# Autodesk Inventor assembly: frame TOPLEVEL
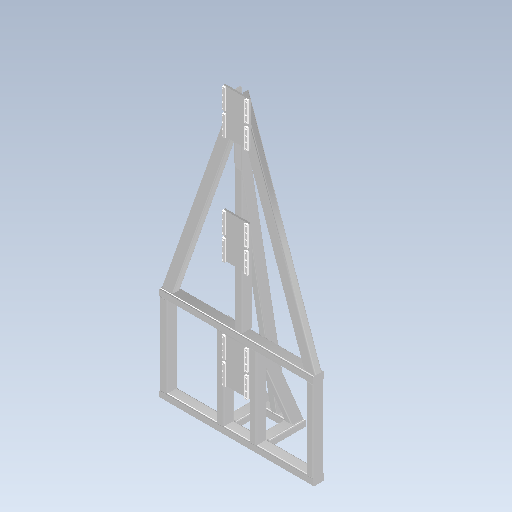
[picture p0: Inventor's stored thumbnail of the model, 512x512]
Saved by Autodesk Inventor 2021 (Build 250183000, 183)
## iProperties
Created: 2021-03-29
Part Number: frame TOPLEVEL
Document SubType Name: Assembly
Designer: Work
Author: Work
## Documents named in this file (12)
- C:\Users\Work\OneDrive - Brookhaven National Laboratory\Daniels, William intern HPR station\Frame\frame TOPLEVEL.iam
- C:\Users\Work\OneDrive - Brookhaven National Laboratory\Daniels, William intern HPR station\Frame\base bar.ipt
- C:\Users\Work\OneDrive - Brookhaven National Laboratory\Daniels, William intern HPR station\Frame\end cap.ipt
- C:\Users\Work\OneDrive - Brookhaven National Laboratory\Daniels, William intern HPR station\Frame\actuMount.iam
- C:\Users\Work\OneDrive - Brookhaven National Laboratory\Daniels, William intern HPR station\Frame\vertical bar.ipt
- C:\Users\Work\OneDrive - Brookhaven National Laboratory\Daniels, William intern HPR station\Frame\depth bar.ipt
- C:\Users\Work\OneDrive - Brookhaven National Laboratory\Daniels, William intern HPR station\Frame\back bar.ipt
- C:\Users\Work\OneDrive - Brookhaven National Laboratory\Daniels, William intern HPR station\Frame\support 1.ipt
- C:\Users\Work\OneDrive - Brookhaven National Laboratory\Daniels, William intern HPR station\Frame\support 2.ipt
- C:\Users\Work\OneDrive - Brookhaven National Laboratory\Daniels, William intern HPR station\Frame\vert support.ipt
- C:\Users\Work\OneDrive - Brookhaven National Laboratory\Daniels, William intern HPR station\Frame\side support.ipt
- C:\Users\Work\OneDrive - Brookhaven National Laboratory\Daniels, William intern HPR station\dimensions.xlsx
## Components (22 placed, 10 different names)
1. base bar:1 — Rigid:1, Rigid:2, Slider:1, Slider:2
2. end cap:1 — Rigid:1, Rigid:3
3. end cap:2 — Rigid:2, Rigid:4
4. actuMount:1 [sub-assembly] — Mate:1, Mate:2, Flush:1, Rigid:11, Rigid:13
5. vertical bar:1 — Rigid:3, Rigid:5
6. vertical bar:2 — Slider:1, Rigid:8, Mate:4, Flush:2
7. vertical bar:3 — Slider:2, Mate:2, Rigid:9, Mate:6, Flush:3
8. vertical bar:4 — Rigid:4, Rigid:6
9. end cap:3 — Rigid:5
10. end cap:4 — Rigid:6, Rigid:7, Mate:12
11. base bar:2 — Rigid:7, Mate:1, Flush:1, Mate:9
12. depth bar:1 — Rigid:8, Rigid:10, Mate:3
13. depth bar:2 — Rigid:9, Mate:5
14. back bar:1 — Rigid:10
15. support 1:1 — Mate:3, Mate:4, Flush:2
16. support 1:2 — Mate:5, Mate:6, Flush:3
17. support 2:1 — Rigid:12, Mate:8, Flush:4, Mate:10, Mate:13
18. actuMount:2 [sub-assembly] — Rigid:11, Rigid:12, Mate:11, Mate:14
19. actuMount:3 [sub-assembly] — Rigid:13, Mate:7
20. vert support:1 — Mate:7, Mate:8, Flush:4
21. side support:1 — Mate:12, Mate:13, Mate:14
22. side support:2 — Mate:9, Mate:10, Mate:11
## Relationships (33: Mate 14, WeldJoint 13, Flush 4, TranslationJoint 2)
- Rigid:1 [WeldJoint]: base bar:1 ↔ end cap:1
- Rigid:2 [WeldJoint]: base bar:1 ↔ end cap:2
- Rigid:3 [WeldJoint]: end cap:1 ↔ vertical bar:1
- Rigid:4 [WeldJoint]: end cap:2 ↔ vertical bar:4
- Slider:1 [TranslationJoint]: base bar:1 ↔ vertical bar:2
- Slider:2 [TranslationJoint]: base bar:1 ↔ vertical bar:3
- Rigid:5 [WeldJoint]: vertical bar:1 ↔ end cap:3
- Rigid:6 [WeldJoint]: vertical bar:4 ↔ end cap:4
- Rigid:7 [WeldJoint]: end cap:4 ↔ base bar:2
- Mate:1: actuMount:1 ↔ base bar:2
- Mate:2: actuMount:1 ↔ vertical bar:3
- Flush:1: actuMount:1 ↔ base bar:2
- Rigid:8 [WeldJoint]: vertical bar:2 ↔ depth bar:1
- Rigid:9 [WeldJoint]: vertical bar:3 ↔ depth bar:2
- Rigid:10 [WeldJoint]: depth bar:1 ↔ back bar:1
- Mate:3: depth bar:1 ↔ support 1:1
- Mate:4: vertical bar:2 ↔ support 1:1
- Flush:2: vertical bar:2 ↔ support 1:1
- Mate:5: depth bar:2 ↔ support 1:2
- Mate:6: vertical bar:3 ↔ support 1:2
- Flush:3: vertical bar:3 ↔ support 1:2
- Rigid:11 [WeldJoint] (-1495.2 mm): actuMount:1 ↔ actuMount:2
- Rigid:12 [WeldJoint]: support 2:1 ↔ actuMount:2
- Rigid:13 [WeldJoint] (-747.6 mm): actuMount:1 ↔ actuMount:3
- Mate:7: actuMount:3 ↔ vert support:1
- Mate:8: support 2:1 ↔ vert support:1
- Flush:4: support 2:1 ↔ vert support:1
- Mate:9: base bar:2 ↔ side support:2
- Mate:10: support 2:1 ↔ side support:2
- Mate:11: actuMount:2 ↔ side support:2
- Mate:12: end cap:4 ↔ side support:1
- Mate:13: support 2:1 ↔ side support:1
- Mate:14: actuMount:2 ↔ side support:1
## Named parameters: height = 203.2 mm, shaftDiam = 6.35 mm, shaftSpace = 1.5875 mm, stageSpace = 2.54 mm, stageAngle = 15 deg, stockHeight = 50.8 mm, stockWidth = 76.2 mm, stockRad = 9.525 mm, stockGuage = 3.175 mm, actuHieght = 1800 mm, groundActu = 304.8 mm, baseWidth = 1066.8 mm, baseDepth = 254 mm, capThickness = 3.175 mm, sup1Len = 660.4 mm, sup1Ang = 22.619865 deg, sup2Len = 2079.37366 mm, sup2Ang = 8.959949 deg, supVertLen = 955.13561 mm, supSideAng = 19.376933 deg, supSideLen = 1531.12879 mm, FlangeDiam = 12.7 mm, bearingDiam = 9.5504 mm, FlangeDepth = 1.5875 mm, smallFilet = 0.39687 mm, thickness = 12.7 mm
